# Autodesk Inventor assembly: LINEAR_INTAKE_ASSY
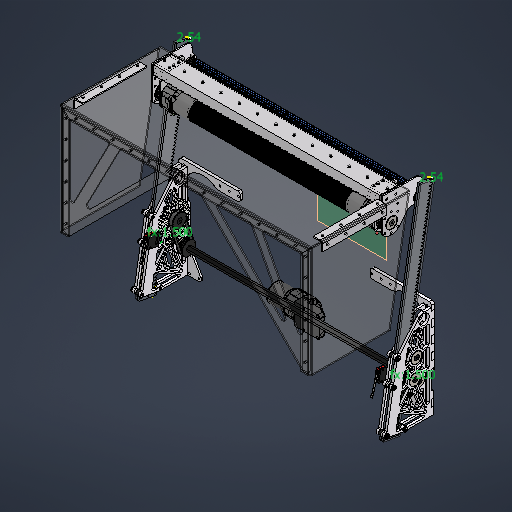
[picture p0: Inventor's stored thumbnail of the model, 512x512]
Saved by Autodesk Inventor 2026 (Build 300175000, 175)
## iProperties
Created: 2026-04-01
Part Number: LINEAR_INTAKE_ASSY
Document SubType Name: Assembly
Designer: 4aida
Mass: 10797 g
Surface Area: 25753.5 cm^2
Volume: 4543.31 cm^3
Density: 2.37645 g/cm^3
Author: 4aida
## Documents named in this file (44)
- C:\Users\littl\OneDrive\Documents\GitHub\2026-Robot-Mechanical\LINEAR_INTAKE\LINEAR_INTAKE_ASSY.iam
- C:\Users\littl\OneDrive\Documents\GitHub\2026-Robot-Mechanical\LINEAR_INTAKE\0.5_Jack_Shaft.ipt
- C:\Users\littl\OneDrive\Documents\GitHub\2026-Robot-Mechanical\#1_CAD Library\Electronics\CONTROLS,SPARK_FLEX.ipt
- C:\Users\littl\OneDrive\Documents\GitHub\2026-Robot-Mechanical\#1_CAD Library\Motors\MOTOR,REV,NEO,VORTEX.ipt
- C:\Users\littl\OneDrive\Documents\GitHub\2026-Robot-Mechanical\LINEAR_INTAKE\RACK_LINEARINTAKE.ipt
- C:\Users\littl\OneDrive\Documents\GitHub\2026-Robot-Mechanical\LINEAR_INTAKE\10DP_Pinion Gear.iam
- C:\Users\littl\OneDrive\Documents\GitHub\2026-Robot-Mechanical\#1_CAD Library\Power Transmission\Bearings\PURCHASED,HEX_BEARING.ipt
- C:\Users\littl\OneDrive\Documents\GitHub\2026-Robot-Mechanical\LINEAR_INTAKE\INTAKE_OUTSIDE_PLATE.ipt
- C:\Users\littl\OneDrive\Documents\GitHub\2026-Robot-Mechanical\LINEAR_INTAKE\RACK_GUIDES.ipt
- C:\Users\littl\OneDrive\Documents\GitHub\2026-Robot-Mechanical\LINEAR_INTAKE\CAST,2inOD,ROLLER.ipt
- C:\Users\littl\OneDrive\Documents\GitHub\2026-Robot-Mechanical\LINEAR_INTAKE\10dp_Ratio_Gears_INTAKE.iam
- C:\Users\littl\OneDrive\Documents\GitHub\2026-Robot-Mechanical\LINEAR_INTAKE\INTAKE_EXT_PULLYS.ipt
- C:\Users\littl\OneDrive\Documents\GitHub\2026-Robot-Mechanical\LINEAR_INTAKE\55t_Belt.ipt
- C:\Users\littl\OneDrive\Documents\GitHub\2026-Robot-Mechanical\LINEAR_INTAKE\12mm_OD_BEARING.ipt
- C:\Users\littl\OneDrive\Documents\GitHub\2026-Robot-Mechanical\LINEAR_INTAKE\fastenal_1140891.ipt
- C:\Users\littl\OneDrive\Documents\GitHub\2026-Robot-Mechanical\LINEAR_INTAKE\SINGLE_BEARING_SPACER.ipt
- C:\Users\littl\OneDrive\Documents\GitHub\2026-Robot-Mechanical\LINEAR_INTAKE\double_BEARING_SPACER.ipt
- C:\Users\littl\OneDrive\Documents\GitHub\2026-Robot-Mechanical\LINEAR_INTAKE\INTAKE_SWERVE_MOUNT.ipt
- C:\Users\littl\OneDrive\Documents\GitHub\2026-Robot-Mechanical\LINEAR_INTAKE\MOUTER_MOUNT_INTAKE.ipt
- C:\Users\littl\OneDrive\Documents\GitHub\2026-Robot-Mechanical\LINEAR_INTAKE\INTAKE_INSIDE_PLATE.ipt
- C:\Users\littl\OneDrive\Documents\GitHub\2026-Robot-Mechanical\LINEAR_INTAKE\INTAKE_BACK_MOUNT_PLATE.ipt
- C:\Users\littl\OneDrive\Documents\GitHub\2026-Robot-Mechanical\LINEAR_INTAKE\PULLY_HEX_SHAFT_INTAKE.ipt
- C:\Users\littl\OneDrive\Documents\GitHub\2026-Robot-Mechanical\LINEAR_INTAKE\PINION_SHAFT_INTAKE.ipt
- C:\Users\littl\OneDrive\Documents\GitHub\2026-Robot-Mechanical\LINEAR_INTAKE\TETHLON_TAPE.ipt
- C:\Users\littl\OneDrive\Documents\GitHub\2026-Robot-Mechanical\LINEAR_INTAKE\PINION_SPACER_INTAKE.ipt
- C:\Users\littl\OneDrive\Documents\GitHub\2026-Robot-Mechanical\LINEAR_INTAKE\PULLY_SPACER_INTAKE.ipt
- C:\Users\littl\OneDrive\Documents\GitHub\2026-Robot-Mechanical\LINEAR_INTAKE\1.25IN Roller.iam
- C:\Users\littl\OneDrive\Documents\GitHub\2026-Robot-Mechanical\LINEAR_INTAKE\CRASH_BAR_INTAKE.ipt
- C:\Users\littl\OneDrive\Documents\GitHub\2026-Robot-Mechanical\LINEAR_INTAKE\TUBE_PLUGS.ipt
- C:\Users\littl\OneDrive\Documents\GitHub\2026-Robot-Mechanical\#1_CAD Library\Electronics\CONTROLS,LIMIT_SWITCH,VEX.iam
- C:\Users\littl\OneDrive\Documents\GitHub\2026-Robot-Mechanical\LINEAR_INTAKE\INSIDE_INTAKE_PLATE.ipt
- C:\Users\littl\OneDrive\Documents\GitHub\2026-Robot-Mechanical\LINEAR_INTAKE\FRONT_INTAKE_LEXAN.ipt
- C:\Users\littl\OneDrive\Documents\GitHub\2026-Robot-Mechanical\LINEAR_INTAKE\SIDE_INTAKE_LEXAN.ipt
- C:\Users\littl\OneDrive\Documents\GitHub\2026-Robot-Mechanical\LINEAR_INTAKE\SIDE_INTAKE_LEXAN_MIR.ipt
- C:\Users\littl\OneDrive\Documents\GitHub\2026-Robot-Mechanical\LINEAR_INTAKE\TOP_INTAKE_LEXAN.ipt
- C:\Users\littl\OneDrive\Documents\GitHub\2026-Robot-Mechanical\LINEAR_INTAKE\LEXAN_CORNER_MOUNT.ipt
- C:\Users\littl\OneDrive\Documents\GitHub\2026-Robot-Mechanical\LINEAR_INTAKE\0.5_Bottom_INTAKE_SHAFT.ipt
- C:\Users\littl\OneDrive\Documents\GitHub\2026-Robot-Mechanical\LINEAR_INTAKE\INTAKE_DRIVER_PULLY.ipt
- C:\Users\littl\OneDrive\Documents\GitHub\2026-Robot-Mechanical\LINEAR_INTAKE\INTAKE_DRIVEN_PULLY.ipt
- C:\Users\littl\OneDrive\Documents\GitHub\2026-Robot-Mechanical\LINEAR_INTAKE\CUT_1.25_Roller.ipt
- C:\Users\littl\OneDrive\Documents\GitHub\2026-Robot-Mechanical\LINEAR_INTAKE\INSIDE_INTAKE_PLATE_MOTOR_MOUNT.ipt
- C:\Users\littl\OneDrive\Documents\GitHub\2026-Robot-Mechanical\LINEAR_INTAKE\CUT_2in_Roller.ipt
- C:\Users\littl\OneDrive\Documents\GitHub\2026-Robot-Mechanical\#1_CAD Library\Building Materials\Fasteners\Bolts\PURCHASED,10-32x0.5in,BUTTONHEAD,BOLT.ipt
- C:\Users\littl\OneDrive\Documents\GitHub\2026-Robot-Mechanical\LINEAR_INTAKE\INSIDE_INTAKE_PLATE_MOTOR_MOUNT_MIR.ipt
## Components (128 placed, 43 different names)
1. RACK_LINEARINTAKE:1 — Mate:149, Mate:230
2. 10DP_Pinion Gear:1 [sub-assembly] — Mate:19, Mate:201
3. INTAKE_OUTSIDE_PLATE:1 — Mate:66, Mate:67, Insert:3, Mate:121, Mate:122, Mate:123, Mate:124, Mate:125, Mate:126, Mate:128, Mate:129, Insert:4, Insert:5, Insert:6, Insert:7, Insert:8, Insert:9, Flush:27, Flush:28, Mate:169, Flush:31, Flush:39, Mate:200, Flush:40
4. INTAKE_OUTSIDE_PLATE:2 — Flush:18, Mate:60, Mate:63, Insert:1, Mate:131, Flush:30, Insert:21, Insert:22, Insert:23, Insert:24, Insert:25, Insert:27, Mate:171, Mate:174, Flush:37, Mate:196, Mate:198, Flush:42, Mate:316, Mate:317, Angle:9
5. RACK_LINEARINTAKE:2
6. 10DP_Pinion Gear:2 [sub-assembly] — Mate:19, Mate:195
7. RACK_GUIDES:1 — Mate:272, Angle:5, Flush:56, Mate:330
8. RACK_GUIDES:4 — Flush:18, Mate:196
9. PURCHASED,HEX_BEARING:3 — Mate:60, Mate:63, Mate:194, Mate:195, Mate:203, Mate:204
10. PURCHASED,HEX_BEARING:4 — Mate:106, Mate:177, Mate:178, Mate:192
11. PURCHASED,HEX_BEARING:5 — Mate:96, Mate:154, Mate:157
12. PURCHASED,HEX_BEARING:6 — Mate:66, Mate:67, Mate:189, Flush:34, Mate:190, Mate:202
13. PURCHASED,HEX_BEARING:7 — Mate:107, Mate:115, Mate:176, Mate:179, Mate:180, Mate:185
14. PURCHASED,HEX_BEARING:10 — Insert:1, Mate:184
15. PURCHASED,HEX_BEARING:11 — Mate:94, Mate:95, Mate:155, Mate:156
16. PURCHASED,HEX_BEARING:12 — Insert:3, Mate:188
17. 10dp_Ratio_Gears_INTAKE:3 [sub-assembly] — Mate:94, Mate:95, Mate:96, Mate:97, Mate:98, Mate:154, Mate:191
18. INTAKE_EXT_PULLYS:5 — Mate:97, Mate:98, Flush:33, Mate:186, Mate:187, Mate:319
19. 10dp_Ratio_Gears_INTAKE:4 [sub-assembly] — Mate:106, Mate:107, Mate:108, Mate:109, Flush:35, Mate:193
20. INTAKE_EXT_PULLYS:7 — Mate:108, Mate:109, Mate:115, Flush:32, Mate:183
21. 12mm_OD_BEARING:1 — Mate:121, Mate:124, Insert:13
22. 12mm_OD_BEARING:2 — Mate:119, Mate:120
23. 12mm_OD_BEARING:3 — Mate:125, Insert:11
24. 12mm_OD_BEARING:4 — Mate:122, Mate:123, Insert:15
25. 12mm_OD_BEARING:5 — Mate:119, Mate:120, Insert:10
26. 12mm_OD_BEARING:6 — Mate:126, Insert:12
27. 12mm_OD_BEARING:12 — Mate:128, Mate:129, Insert:14
28. fastenal_1140891:1 — Insert:4
29. fastenal_1140891:2 — Insert:5
30. fastenal_1140891:3 — Insert:8
31. fastenal_1140891:4 — Insert:9
32. fastenal_1140891:5 — Insert:7
33. fastenal_1140891:6 — Insert:6
34. SINGLE_BEARING_SPACER:3 — Insert:10
35. double_BEARING_SPACER:1 — Insert:11
36. double_BEARING_SPACER:2 — Insert:15
37. double_BEARING_SPACER:3 — Insert:12
38. double_BEARING_SPACER:4 — Insert:13
39. double_BEARING_SPACER:5 — Insert:14
40. INTAKE_SWERVE_MOUNT:1 — Flush:27, Flush:28, Flush:29, Mate:150, Mate:318
41. INTAKE_SWERVE_MOUNT:2 — Mate:131, Flush:29, Flush:30, Mate:172, Mate:181
42. 12mm_OD_BEARING:13 — Mate:135, Mate:136
43. fastenal_1140891:7 — Mate:135, Mate:136, Insert:24
44. double_BEARING_SPACER:6
45. 12mm_OD_BEARING:14
46. fastenal_1140891:8 — Insert:25
47. double_BEARING_SPACER:7
48. 12mm_OD_BEARING:15
49. fastenal_1140891:9 — Insert:23
50. double_BEARING_SPACER:8
51. 12mm_OD_BEARING:16
52. fastenal_1140891:10 — Insert:21
53. double_BEARING_SPACER:9
54. 12mm_OD_BEARING:17
55. fastenal_1140891:11 — Insert:22
56. double_BEARING_SPACER:10
57. 12mm_OD_BEARING:18
58. 12mm_OD_BEARING:19 — Mate:147
59. fastenal_1140891:12 — Mate:147, Mate:148, Insert:27
60. SINGLE_BEARING_SPACER:4 — Mate:148
61. INTAKE_INSIDE_PLATE:1 — Mate:149, Mate:150, Mate:155, Mate:156, Mate:157, Mate:168, Flush:38, Mate:199, Flush:41, Mate:289, Mate:290, Mate:291, Mate:292, Mate:300, Mate:318
62. INTAKE_BACK_MOUNT_PLATE:1 — Mate:168, Mate:169, Flush:31
63. INTAKE_BACK_MOUNT_PLATE:2 — Mate:171, Mate:315, Mate:316, Mate:317
64. INTAKE_INSIDE_PLATE:3 — Mate:172, Mate:174, Mate:176, Mate:177, Mate:178, Mate:179, Mate:180, Mate:181, Flush:36, Mate:197, Flush:43, Mate:286, Mate:287, Mate:288, Insert:28, Angle:6
65. PULLY_HEX_SHAFT_INTAKE:1 — Flush:32, Mate:183, Mate:184, Mate:185
66. PULLY_HEX_SHAFT_INTAKE:2 — Flush:33, Mate:186, Mate:187, Mate:188
67. PINION_SHAFT_INTAKE:1 — Mate:189, Flush:34, Mate:190, Mate:191
68. PINION_SHAFT_INTAKE:2 — Mate:192, Flush:35, Mate:193, Mate:194
69. TETHLON_TAPE:1 — Flush:36, Mate:197, Flush:43
70. TETHLON_TAPE:2 — Flush:38, Mate:198, Flush:42
71. TETHLON_TAPE:3 — Flush:37, Mate:200, Flush:40
72. TETHLON_TAPE:4 — Flush:39, Mate:199, Flush:41
73. PINION_SPACER_INTAKE:1 — Mate:203, Mate:204
74. PINION_SPACER_INTAKE:2 — Mate:201, Mate:202
75. CRASH_BAR_INTAKE:1 — Mate:220, Mate:224, Mate:225, Mate:226, Mate:227, Mate:228, Mate:229, Mate:230, Mate:274, Flush:55, Mate:330, Mate:373, Mate:374, Mate:386
76. TUBE_PLUGS:1 — Mate:227, Mate:228, Mate:229, Mate:235, Mate:236, Mate:263
77. TUBE_PLUGS:2 — Mate:224, Mate:225, Mate:226, Mate:231, Mate:232, Mate:233
78. INSIDE_INTAKE_PLATE:1 — Mate:231, Mate:232, Mate:233, Mate:242, Mate:327, Mate:328, Mate:335, Insert:29, Angle:7, Mate:385
79. 1.25IN Roller:6 [sub-assembly] — Mate:242, Mate:253, Mate:254, Flush:49, Mate:370
80. INSIDE_INTAKE_PLATE:2 — Mate:235, Mate:236, Mate:263, Mate:325, Mate:326, Mate:337, Mate:338, Angle:8, Mate:383
81. CAST,2inOD,ROLLER:9 — Mate:264, Mate:267, Mate:379
82. 1.25IN Roller:7 [sub-assembly] — Mate:253, Mate:254, Mate:255, Mate:256, Flush:49, Flush:50, Flush:51
83. 1.25IN Roller:8 [sub-assembly] — Mate:255, Mate:256, Flush:50, Mate:257, Mate:258, Flush:51
84. 1.25IN Roller:9 [sub-assembly] — Mate:257, Mate:258, Mate:371
85. CAST,2inOD,ROLLER:10 — Mate:264, Mate:265, Mate:267, Mate:268
86. CAST,2inOD,ROLLER:11 — Mate:265, Mate:268, Mate:367, Mate:368, Mate:369, Mate:380
87. FRONT_INTAKE_LEXAN:2 — Mate:274, Flush:55, Flush:56, Mate:275, Mate:276, Flush:57, Mate:277, Flush:58, Mate:278, Flush:60, Mate:280, Mate:282, Mate:285, Angle:9
88. SIDE_INTAKE_LEXAN:1 — Mate:275, Mate:276, Flush:57, Mate:281
89. SIDE_INTAKE_LEXAN_MIR:1 — Mate:277, Flush:58, Mate:278, Mate:279, Flush:59, Mate:283, Mate:284
90. TOP_INTAKE_LEXAN:1 — Mate:279, Flush:59, Flush:60
91. LEXAN_CORNER_MOUNT:1 — Mate:280, Mate:281, Mate:285
92. LEXAN_CORNER_MOUNT:2 — Mate:282, Mate:283, Mate:284
93. CONTROLS,LIMIT_SWITCH,VEX:2 [sub-assembly] — Mate:286, Mate:287, Mate:288
94. CONTROLS,LIMIT_SWITCH,VEX:3 [sub-assembly] — Mate:289, Mate:290, Mate:291
95. PURCHASED,HEX_BEARING:16 — Mate:292, Mate:294, Mate:299, Mate:300, Flush:61, Mate:321
96. 55t_Belt:3 — Mate:294, Mate:295, Mate:296, Mate:319
97. INTAKE_EXT_PULLYS:10 — Mate:295, Mate:296, Mate:297, Mate:298, Mate:301, Mate:324
98. PULLY_SPACER_INTAKE:3 — Mate:297, Mate:298, Mate:299
99. 0.5_Jack_Shaft:4 — Mate:301, Mate:320, Flush:61, Mate:321, Mate:322, Flush:62, Mate:323, Mate:324
100. PURCHASED,HEX_BEARING:17 — Insert:28, Mate:320, Flush:62, Mate:323
101. INTAKE_EXT_PULLYS:11 — Mate:305, Mate:307, Mate:308, Mate:322
102. PULLY_SPACER_INTAKE:4 — Mate:305
103. 55t_Belt:4 — Mate:307, Mate:308
104. CONTROLS,SPARK_FLEX:6
105. MOTOR,REV,NEO,VORTEX:6
106. MOUTER_MOUNT_INTAKE:2 — Mate:315, Angle:6
107. PURCHASED,HEX_BEARING:18 — Mate:325, Mate:326, Flush:63, Mate:331, Mate:363, Mate:364, Mate:365, Mate:382
108. PURCHASED,HEX_BEARING:19 — Mate:327, Mate:328, Mate:359, Mate:360, Mate:361, Mate:384
109. 0.5_Bottom_INTAKE_SHAFT:1 — Flush:63, Mate:331, Mate:359, Mate:362, Mate:364, Mate:366
110. CONTROLS,SPARK_FLEX:7 — Mate:356, Angle:7, Mate:388
111. MOTOR,REV,NEO,VORTEX:7 — Mate:357, Mate:379, Mate:387
112. 0.5_Bottom_INTAKE_SHAFT:2 — Mate:335, Flush:64, Mate:336, Mate:339, Mate:347, Mate:348, Mate:353, Mate:354, Mate:367, Mate:368, Mate:369
113. PURCHASED,HEX_BEARING:20 — Insert:29, Flush:64, Mate:336, Mate:343, Mate:344, Mate:350
114. PURCHASED,HEX_BEARING:21 — Mate:337, Mate:338, Mate:339, Mate:345, Mate:346
115. CONTROLS,SPARK_FLEX:8 — Mate:355, Angle:8, Mate:375
116. MOTOR,REV,NEO,VORTEX:8 — Mate:358, Mate:381
117. INTAKE_DRIVER_PULLY:1 — Mate:343, Mate:344, Mate:348, Mate:349
118. INTAKE_DRIVER_PULLY:2 — Mate:345, Mate:346, Mate:347, Mate:351, Mate:352
119. PURCHASED,HEX_BEARING:22 — Mate:349, Mate:350, Mate:354, Mate:356, Mate:357
120. PURCHASED,HEX_BEARING:23 — Mate:351, Mate:352, Mate:353, Mate:355, Mate:358
121. INTAKE_DRIVEN_PULLY:1 — Mate:360, Mate:361, Mate:362, Mate:370
122. INTAKE_DRIVEN_PULLY:2 — Mate:363, Mate:365, Mate:366, Mate:372
123. CUT_1.25_Roller:1 — Mate:371, Mate:372
124. INSIDE_INTAKE_PLATE_MOTOR_MOUNT:1 — Mate:373, Mate:374, Mate:375
125. CUT_2in_Roller:1 — Mate:380, Mate:381
126. PURCHASED,10-32x0.5in,BUTTONHEAD,BOLT:1 — Mate:382, Mate:383
127. PURCHASED,10-32x0.5in,BUTTONHEAD,BOLT:2 — Mate:384, Mate:385
128. INSIDE_INTAKE_PLATE_MOTOR_MOUNT_MIR:1 — Mate:386, Mate:387, Mate:388
## Relationships (290: Mate 217, Flush 40, Insert 28, Angle 5)
- [Flush]: RACK_LINEARINTAKE:1 ↔ 10DP_Pinion Gear:1
- [Flush] (6 mm): RACK_LINEARINTAKE:1 ↔ INTAKE_OUTSIDE_PLATE:1
- [Mate] (5.2705 mm): RACK_LINEARINTAKE:1 ↔ INTAKE_OUTSIDE_PLATE:1
- [Flush]: RACK_LINEARINTAKE:2 ↔ 10DP_Pinion Gear:2
- [Flush]: RACK_LINEARINTAKE:1 ↔ RACK_LINEARINTAKE:2
- [Flush]: RACK_LINEARINTAKE:1 ↔ RACK_LINEARINTAKE:2
- Mate:19: 10DP_Pinion Gear:1 ↔ 10DP_Pinion Gear:2
- [Mate]: RACK_LINEARINTAKE:1 ↔ RACK_GUIDES:1
- [Mate]: RACK_LINEARINTAKE:2 ↔ RACK_GUIDES:4
- [Flush]: RACK_LINEARINTAKE:2 ↔ RACK_GUIDES:4
- [Flush]: RACK_LINEARINTAKE:2 ↔ RACK_GUIDES:4
- [Flush]: RACK_LINEARINTAKE:1 ↔ RACK_GUIDES:1
- [Flush]: RACK_LINEARINTAKE:1 ↔ RACK_GUIDES:1
- Flush:18: INTAKE_OUTSIDE_PLATE:2 ↔ RACK_GUIDES:4
- Mate:60: INTAKE_OUTSIDE_PLATE:2 ↔ PURCHASED,HEX_BEARING:3
- Mate:63: INTAKE_OUTSIDE_PLATE:2 ↔ PURCHASED,HEX_BEARING:3
- Mate:66: INTAKE_OUTSIDE_PLATE:1 ↔ PURCHASED,HEX_BEARING:6
- Mate:67: INTAKE_OUTSIDE_PLATE:1 ↔ PURCHASED,HEX_BEARING:6
- Insert:1: INTAKE_OUTSIDE_PLATE:2 ↔ PURCHASED,HEX_BEARING:10
- Insert:3: INTAKE_OUTSIDE_PLATE:1 ↔ PURCHASED,HEX_BEARING:12
- Mate:94: PURCHASED,HEX_BEARING:11 ↔ 10dp_Ratio_Gears_INTAKE:3
- Mate:95: PURCHASED,HEX_BEARING:11 ↔ 10dp_Ratio_Gears_INTAKE:3
- Mate:96: PURCHASED,HEX_BEARING:5 ↔ 10dp_Ratio_Gears_INTAKE:3
- Mate:97: 10dp_Ratio_Gears_INTAKE:3 ↔ INTAKE_EXT_PULLYS:5
- Mate:98: 10dp_Ratio_Gears_INTAKE:3 ↔ INTAKE_EXT_PULLYS:5
- Mate:106: PURCHASED,HEX_BEARING:4 ↔ 10dp_Ratio_Gears_INTAKE:4
- Mate:107: PURCHASED,HEX_BEARING:7 ↔ 10dp_Ratio_Gears_INTAKE:4
- Mate:108: 10dp_Ratio_Gears_INTAKE:4 ↔ INTAKE_EXT_PULLYS:7
- Mate:109: 10dp_Ratio_Gears_INTAKE:4 ↔ INTAKE_EXT_PULLYS:7
- Mate:115: PURCHASED,HEX_BEARING:7 ↔ INTAKE_EXT_PULLYS:7
- Mate:119: 12mm_OD_BEARING:2 ↔ 12mm_OD_BEARING:5
- Mate:120: 12mm_OD_BEARING:2 ↔ 12mm_OD_BEARING:5
- Mate:121: INTAKE_OUTSIDE_PLATE:1 ↔ 12mm_OD_BEARING:1
- Mate:122: INTAKE_OUTSIDE_PLATE:1 ↔ 12mm_OD_BEARING:4
- Mate:123: INTAKE_OUTSIDE_PLATE:1 ↔ 12mm_OD_BEARING:4
- Mate:124: INTAKE_OUTSIDE_PLATE:1 ↔ 12mm_OD_BEARING:1
- Mate:125: INTAKE_OUTSIDE_PLATE:1 ↔ 12mm_OD_BEARING:3
- Mate:126: INTAKE_OUTSIDE_PLATE:1 ↔ 12mm_OD_BEARING:6
- Mate:128: INTAKE_OUTSIDE_PLATE:1 ↔ 12mm_OD_BEARING:12
- Mate:129: INTAKE_OUTSIDE_PLATE:1 ↔ 12mm_OD_BEARING:12
- Insert:4: INTAKE_OUTSIDE_PLATE:1 ↔ fastenal_1140891:1
- Insert:5: INTAKE_OUTSIDE_PLATE:1 ↔ fastenal_1140891:2
- Insert:6: INTAKE_OUTSIDE_PLATE:1 ↔ fastenal_1140891:6
- Insert:7: INTAKE_OUTSIDE_PLATE:1 ↔ fastenal_1140891:5
- Insert:8: INTAKE_OUTSIDE_PLATE:1 ↔ fastenal_1140891:3
- Insert:9: INTAKE_OUTSIDE_PLATE:1 ↔ fastenal_1140891:4
- Insert:10: 12mm_OD_BEARING:5 ↔ SINGLE_BEARING_SPACER:3
- Insert:11: 12mm_OD_BEARING:3 ↔ double_BEARING_SPACER:1
- Insert:12: 12mm_OD_BEARING:6 ↔ double_BEARING_SPACER:3
- Insert:13: 12mm_OD_BEARING:1 ↔ double_BEARING_SPACER:4
- Insert:14: 12mm_OD_BEARING:12 ↔ double_BEARING_SPACER:5
- Insert:15: 12mm_OD_BEARING:4 ↔ double_BEARING_SPACER:2
- Flush:27: INTAKE_OUTSIDE_PLATE:1 ↔ INTAKE_SWERVE_MOUNT:1
- Flush:28 (-12.2199 mm): INTAKE_OUTSIDE_PLATE:1 ↔ INTAKE_SWERVE_MOUNT:1
- Mate:131: INTAKE_OUTSIDE_PLATE:2 ↔ INTAKE_SWERVE_MOUNT:2
- Flush:29: INTAKE_SWERVE_MOUNT:1 ↔ INTAKE_SWERVE_MOUNT:2
- Flush:30: INTAKE_OUTSIDE_PLATE:2 ↔ INTAKE_SWERVE_MOUNT:2
- [Insert]: 12mm_OD_BEARING:13 ↔ double_BEARING_SPACER:6
- Mate:135 (6.35 mm): 12mm_OD_BEARING:13 ↔ fastenal_1140891:7
- Mate:136: 12mm_OD_BEARING:13 ↔ fastenal_1140891:7
- [Insert]: 12mm_OD_BEARING:14 ↔ double_BEARING_SPACER:7
- [Mate] (6.35 mm): 12mm_OD_BEARING:14 ↔ fastenal_1140891:8
- [Mate]: 12mm_OD_BEARING:14 ↔ fastenal_1140891:8
- [Insert]: 12mm_OD_BEARING:15 ↔ double_BEARING_SPACER:8
- [Mate] (6.35 mm): 12mm_OD_BEARING:15 ↔ fastenal_1140891:9
- [Mate]: 12mm_OD_BEARING:15 ↔ fastenal_1140891:9
- [Insert]: 12mm_OD_BEARING:16 ↔ double_BEARING_SPACER:9
- [Mate] (6.35 mm): 12mm_OD_BEARING:16 ↔ fastenal_1140891:10
- [Mate]: 12mm_OD_BEARING:16 ↔ fastenal_1140891:10
- [Insert]: 12mm_OD_BEARING:17 ↔ double_BEARING_SPACER:10
- [Mate] (6.35 mm): 12mm_OD_BEARING:17 ↔ fastenal_1140891:11
- [Mate]: 12mm_OD_BEARING:17 ↔ fastenal_1140891:11
- Insert:21: INTAKE_OUTSIDE_PLATE:2 ↔ fastenal_1140891:10
- Insert:22: INTAKE_OUTSIDE_PLATE:2 ↔ fastenal_1140891:11
- Insert:23: INTAKE_OUTSIDE_PLATE:2 ↔ fastenal_1140891:9
- Insert:24: INTAKE_OUTSIDE_PLATE:2 ↔ fastenal_1140891:7
- Insert:25: INTAKE_OUTSIDE_PLATE:2 ↔ fastenal_1140891:8
- [Mate]: 12mm_OD_BEARING:18 ↔ 12mm_OD_BEARING:19
- [Mate]: 12mm_OD_BEARING:18 ↔ 12mm_OD_BEARING:19
- [Insert]: 12mm_OD_BEARING:19 ↔ SINGLE_BEARING_SPACER:4
- Mate:147: 12mm_OD_BEARING:19 ↔ fastenal_1140891:12
- Mate:148 (6.35 mm): fastenal_1140891:12 ↔ SINGLE_BEARING_SPACER:4
- Insert:27: INTAKE_OUTSIDE_PLATE:2 ↔ fastenal_1140891:12
- Mate:149 (0.508 mm): RACK_LINEARINTAKE:1 ↔ INTAKE_INSIDE_PLATE:1
- Mate:150: INTAKE_SWERVE_MOUNT:1 ↔ INTAKE_INSIDE_PLATE:1
- Mate:154: PURCHASED,HEX_BEARING:5 ↔ 10dp_Ratio_Gears_INTAKE:3
- Mate:155: PURCHASED,HEX_BEARING:11 ↔ INTAKE_INSIDE_PLATE:1
- Mate:156: PURCHASED,HEX_BEARING:11 ↔ INTAKE_INSIDE_PLATE:1
- Mate:157: PURCHASED,HEX_BEARING:5 ↔ INTAKE_INSIDE_PLATE:1
- Mate:168: INTAKE_INSIDE_PLATE:1 ↔ INTAKE_BACK_MOUNT_PLATE:1
- Mate:169: INTAKE_OUTSIDE_PLATE:1 ↔ INTAKE_BACK_MOUNT_PLATE:1
- Flush:31: INTAKE_OUTSIDE_PLATE:1 ↔ INTAKE_BACK_MOUNT_PLATE:1
- Mate:171: INTAKE_OUTSIDE_PLATE:2 ↔ INTAKE_BACK_MOUNT_PLATE:2
- Mate:172: INTAKE_SWERVE_MOUNT:2 ↔ INTAKE_INSIDE_PLATE:3
- Mate:174: INTAKE_OUTSIDE_PLATE:2 ↔ INTAKE_INSIDE_PLATE:3
- Mate:176: PURCHASED,HEX_BEARING:7 ↔ INTAKE_INSIDE_PLATE:3
- Mate:177: PURCHASED,HEX_BEARING:4 ↔ INTAKE_INSIDE_PLATE:3
- Mate:178: PURCHASED,HEX_BEARING:4 ↔ INTAKE_INSIDE_PLATE:3
- Mate:179: PURCHASED,HEX_BEARING:7 ↔ INTAKE_INSIDE_PLATE:3
- Mate:180: PURCHASED,HEX_BEARING:7 ↔ INTAKE_INSIDE_PLATE:3
- Mate:181: INTAKE_SWERVE_MOUNT:2 ↔ INTAKE_INSIDE_PLATE:3
- Flush:32: INTAKE_EXT_PULLYS:7 ↔ PULLY_HEX_SHAFT_INTAKE:1
- Mate:183: INTAKE_EXT_PULLYS:7 ↔ PULLY_HEX_SHAFT_INTAKE:1
- Mate:184: PURCHASED,HEX_BEARING:10 ↔ PULLY_HEX_SHAFT_INTAKE:1
- Mate:185: PURCHASED,HEX_BEARING:7 ↔ PULLY_HEX_SHAFT_INTAKE:1
- Flush:33: INTAKE_EXT_PULLYS:5 ↔ PULLY_HEX_SHAFT_INTAKE:2
- Mate:186: INTAKE_EXT_PULLYS:5 ↔ PULLY_HEX_SHAFT_INTAKE:2
- Mate:187: INTAKE_EXT_PULLYS:5 ↔ PULLY_HEX_SHAFT_INTAKE:2
- Mate:188: PURCHASED,HEX_BEARING:12 ↔ PULLY_HEX_SHAFT_INTAKE:2
- Mate:189: PURCHASED,HEX_BEARING:6 ↔ PINION_SHAFT_INTAKE:1
- Flush:34: PURCHASED,HEX_BEARING:6 ↔ PINION_SHAFT_INTAKE:1
- Mate:190: PURCHASED,HEX_BEARING:6 ↔ PINION_SHAFT_INTAKE:1
- Mate:191: 10dp_Ratio_Gears_INTAKE:3 ↔ PINION_SHAFT_INTAKE:1
- Mate:192: PURCHASED,HEX_BEARING:4 ↔ PINION_SHAFT_INTAKE:2
- Flush:35: 10dp_Ratio_Gears_INTAKE:4 ↔ PINION_SHAFT_INTAKE:2
- Mate:193: 10dp_Ratio_Gears_INTAKE:4 ↔ PINION_SHAFT_INTAKE:2
- Mate:194: PURCHASED,HEX_BEARING:3 ↔ PINION_SHAFT_INTAKE:2
- Flush:36: INTAKE_INSIDE_PLATE:3 ↔ TETHLON_TAPE:1
- Flush:37: INTAKE_OUTSIDE_PLATE:2 ↔ TETHLON_TAPE:3
- Flush:38: INTAKE_INSIDE_PLATE:1 ↔ TETHLON_TAPE:2
- Flush:39: INTAKE_OUTSIDE_PLATE:1 ↔ TETHLON_TAPE:4
- Mate:195: 10DP_Pinion Gear:2 ↔ PURCHASED,HEX_BEARING:3
- Mate:196 (0.508 mm): INTAKE_OUTSIDE_PLATE:2 ↔ RACK_GUIDES:4
- Mate:197: INTAKE_INSIDE_PLATE:3 ↔ TETHLON_TAPE:1
- Mate:198: INTAKE_OUTSIDE_PLATE:2 ↔ TETHLON_TAPE:2
- Mate:199: INTAKE_INSIDE_PLATE:1 ↔ TETHLON_TAPE:4
- Mate:200: INTAKE_OUTSIDE_PLATE:1 ↔ TETHLON_TAPE:3
- Flush:40: INTAKE_OUTSIDE_PLATE:1 ↔ TETHLON_TAPE:3
- Flush:41: INTAKE_INSIDE_PLATE:1 ↔ TETHLON_TAPE:4
- Flush:42: INTAKE_OUTSIDE_PLATE:2 ↔ TETHLON_TAPE:2
- Flush:43: INTAKE_INSIDE_PLATE:3 ↔ TETHLON_TAPE:1
- Mate:201: 10DP_Pinion Gear:1 ↔ PINION_SPACER_INTAKE:2
- Mate:202: PURCHASED,HEX_BEARING:6 ↔ PINION_SPACER_INTAKE:2
- Mate:203: PURCHASED,HEX_BEARING:3 ↔ PINION_SPACER_INTAKE:1
- Mate:204: PURCHASED,HEX_BEARING:3 ↔ PINION_SPACER_INTAKE:1
- Mate:220: CRASH_BAR_INTAKE:1
- Mate:224: CRASH_BAR_INTAKE:1 ↔ TUBE_PLUGS:2
- Mate:225: CRASH_BAR_INTAKE:1 ↔ TUBE_PLUGS:2
- Mate:226: CRASH_BAR_INTAKE:1 ↔ TUBE_PLUGS:2
- Mate:227: CRASH_BAR_INTAKE:1 ↔ TUBE_PLUGS:1
- Mate:228: CRASH_BAR_INTAKE:1 ↔ TUBE_PLUGS:1
- Mate:229: CRASH_BAR_INTAKE:1 ↔ TUBE_PLUGS:1
- Mate:230: RACK_LINEARINTAKE:1 ↔ CRASH_BAR_INTAKE:1
- Mate:231: TUBE_PLUGS:2 ↔ INSIDE_INTAKE_PLATE:1
- Mate:232: TUBE_PLUGS:2 ↔ INSIDE_INTAKE_PLATE:1
- Mate:233: TUBE_PLUGS:2 ↔ INSIDE_INTAKE_PLATE:1
- Mate:235: TUBE_PLUGS:1 ↔ INSIDE_INTAKE_PLATE:2
- Mate:236: TUBE_PLUGS:1 ↔ INSIDE_INTAKE_PLATE:2
- Mate:242: INSIDE_INTAKE_PLATE:1 ↔ 1.25IN Roller:6
- Mate:253: 1.25IN Roller:6 ↔ 1.25IN Roller:7
- Mate:254: 1.25IN Roller:6 ↔ 1.25IN Roller:7
- Mate:255: 1.25IN Roller:7 ↔ 1.25IN Roller:8
- Mate:256: 1.25IN Roller:7 ↔ 1.25IN Roller:8
- Flush:49: 1.25IN Roller:6 ↔ 1.25IN Roller:7
- Flush:50: 1.25IN Roller:7 ↔ 1.25IN Roller:8
- Mate:257: 1.25IN Roller:8 ↔ 1.25IN Roller:9
- Mate:258: 1.25IN Roller:8 ↔ 1.25IN Roller:9
- Flush:51: 1.25IN Roller:7 ↔ 1.25IN Roller:8
- Mate:263: TUBE_PLUGS:1 ↔ INSIDE_INTAKE_PLATE:2
- Mate:264: CAST,2inOD,ROLLER:9 ↔ CAST,2inOD,ROLLER:10
- Mate:265: CAST,2inOD,ROLLER:10 ↔ CAST,2inOD,ROLLER:11
- Mate:267: CAST,2inOD,ROLLER:9 ↔ CAST,2inOD,ROLLER:10
- Mate:268: CAST,2inOD,ROLLER:10 ↔ CAST,2inOD,ROLLER:11
- Mate:272: RACK_GUIDES:1
- Angle:5 (10 deg): RACK_GUIDES:1
- Mate:274: CRASH_BAR_INTAKE:1 ↔ FRONT_INTAKE_LEXAN:2
- Flush:55: CRASH_BAR_INTAKE:1 ↔ FRONT_INTAKE_LEXAN:2
- Flush:56 (-3.175 mm): RACK_GUIDES:1 ↔ FRONT_INTAKE_LEXAN:2
- Mate:275: FRONT_INTAKE_LEXAN:2 ↔ SIDE_INTAKE_LEXAN:1
- Mate:276: FRONT_INTAKE_LEXAN:2 ↔ SIDE_INTAKE_LEXAN:1
- Flush:57: FRONT_INTAKE_LEXAN:2 ↔ SIDE_INTAKE_LEXAN:1
- Mate:277: FRONT_INTAKE_LEXAN:2 ↔ SIDE_INTAKE_LEXAN_MIR:1
- Flush:58: FRONT_INTAKE_LEXAN:2 ↔ SIDE_INTAKE_LEXAN_MIR:1
- Mate:278: FRONT_INTAKE_LEXAN:2 ↔ SIDE_INTAKE_LEXAN_MIR:1
- Mate:279: SIDE_INTAKE_LEXAN_MIR:1 ↔ TOP_INTAKE_LEXAN:1
- Flush:59: SIDE_INTAKE_LEXAN_MIR:1 ↔ TOP_INTAKE_LEXAN:1
- Flush:60: FRONT_INTAKE_LEXAN:2 ↔ TOP_INTAKE_LEXAN:1
- Mate:280: FRONT_INTAKE_LEXAN:2 ↔ LEXAN_CORNER_MOUNT:1
- Mate:281: SIDE_INTAKE_LEXAN:1 ↔ LEXAN_CORNER_MOUNT:1
- Mate:282: FRONT_INTAKE_LEXAN:2 ↔ LEXAN_CORNER_MOUNT:2
- Mate:283: SIDE_INTAKE_LEXAN_MIR:1 ↔ LEXAN_CORNER_MOUNT:2
- Mate:284: SIDE_INTAKE_LEXAN_MIR:1 ↔ LEXAN_CORNER_MOUNT:2
- Mate:285: FRONT_INTAKE_LEXAN:2 ↔ LEXAN_CORNER_MOUNT:1
- Mate:286: INTAKE_INSIDE_PLATE:3 ↔ CONTROLS,LIMIT_SWITCH,VEX:2
- Mate:287 (-12.7 mm): INTAKE_INSIDE_PLATE:3 ↔ CONTROLS,LIMIT_SWITCH,VEX:2
- Mate:288: INTAKE_INSIDE_PLATE:3 ↔ CONTROLS,LIMIT_SWITCH,VEX:2
- Mate:289: INTAKE_INSIDE_PLATE:1 ↔ CONTROLS,LIMIT_SWITCH,VEX:3
- Mate:290: INTAKE_INSIDE_PLATE:1 ↔ CONTROLS,LIMIT_SWITCH,VEX:3
- Mate:291: INTAKE_INSIDE_PLATE:1 ↔ CONTROLS,LIMIT_SWITCH,VEX:3
- Mate:292: INTAKE_INSIDE_PLATE:1 ↔ PURCHASED,HEX_BEARING:16
- Mate:294: PURCHASED,HEX_BEARING:16 ↔ 55t_Belt:3
- Mate:295: 55t_Belt:3 ↔ INTAKE_EXT_PULLYS:10
- Mate:296: 55t_Belt:3 ↔ INTAKE_EXT_PULLYS:10
- Mate:297: INTAKE_EXT_PULLYS:10 ↔ PULLY_SPACER_INTAKE:3
- Mate:298: INTAKE_EXT_PULLYS:10 ↔ PULLY_SPACER_INTAKE:3
- Mate:299: PURCHASED,HEX_BEARING:16 ↔ PULLY_SPACER_INTAKE:3
- Mate:300: INTAKE_INSIDE_PLATE:1 ↔ PURCHASED,HEX_BEARING:16
- Mate:301: INTAKE_EXT_PULLYS:10 ↔ 0.5_Jack_Shaft:4
- [Mate]: PURCHASED,HEX_BEARING:17 ↔ INTAKE_EXT_PULLYS:11
- [Mate]: PURCHASED,HEX_BEARING:17 ↔ PULLY_SPACER_INTAKE:4
- [Mate]: PURCHASED,HEX_BEARING:17 ↔ PULLY_SPACER_INTAKE:4
- Insert:28: INTAKE_INSIDE_PLATE:3 ↔ PURCHASED,HEX_BEARING:17
- Mate:305: INTAKE_EXT_PULLYS:11 ↔ PULLY_SPACER_INTAKE:4
- Mate:307: INTAKE_EXT_PULLYS:11 ↔ 55t_Belt:4
- Mate:308: INTAKE_EXT_PULLYS:11 ↔ 55t_Belt:4
- [Mate]: CONTROLS,SPARK_FLEX:6 ↔ MOTOR,REV,NEO,VORTEX:6
- [Mate]: CONTROLS,SPARK_FLEX:6 ↔ MOTOR,REV,NEO,VORTEX:6
- [Mate]: CONTROLS,SPARK_FLEX:6 ↔ MOTOR,REV,NEO,VORTEX:6
- [Mate]: CONTROLS,SPARK_FLEX:6 ↔ MOUTER_MOUNT_INTAKE:2
- [Mate]: MOTOR,REV,NEO,VORTEX:6 ↔ MOUTER_MOUNT_INTAKE:2
- [Mate]: CONTROLS,SPARK_FLEX:6 ↔ MOUTER_MOUNT_INTAKE:2
- Mate:315 (3.175 mm): INTAKE_BACK_MOUNT_PLATE:2 ↔ MOUTER_MOUNT_INTAKE:2
- Mate:316: INTAKE_OUTSIDE_PLATE:2 ↔ INTAKE_BACK_MOUNT_PLATE:2
- Mate:317: INTAKE_OUTSIDE_PLATE:2 ↔ INTAKE_BACK_MOUNT_PLATE:2
- Angle:6 (0 deg): INTAKE_INSIDE_PLATE:3 ↔ MOUTER_MOUNT_INTAKE:2
- Mate:318: INTAKE_SWERVE_MOUNT:1 ↔ INTAKE_INSIDE_PLATE:1
- Mate:319: INTAKE_EXT_PULLYS:5 ↔ 55t_Belt:3
- Mate:320: 0.5_Jack_Shaft:4 ↔ PURCHASED,HEX_BEARING:17
- Flush:61: PURCHASED,HEX_BEARING:16 ↔ 0.5_Jack_Shaft:4
- Mate:321: PURCHASED,HEX_BEARING:16 ↔ 0.5_Jack_Shaft:4
- Mate:322: 0.5_Jack_Shaft:4 ↔ INTAKE_EXT_PULLYS:11
- Flush:62: 0.5_Jack_Shaft:4 ↔ PURCHASED,HEX_BEARING:17
- Mate:323: 0.5_Jack_Shaft:4 ↔ PURCHASED,HEX_BEARING:17
- Mate:324: INTAKE_EXT_PULLYS:10 ↔ 0.5_Jack_Shaft:4
- Mate:325: INSIDE_INTAKE_PLATE:2 ↔ PURCHASED,HEX_BEARING:18
- Mate:326: INSIDE_INTAKE_PLATE:2 ↔ PURCHASED,HEX_BEARING:18
- Mate:327: INSIDE_INTAKE_PLATE:1 ↔ PURCHASED,HEX_BEARING:19
- Mate:328: INSIDE_INTAKE_PLATE:1 ↔ PURCHASED,HEX_BEARING:19
- Mate:330 (-120.8143 mm): RACK_GUIDES:1 ↔ CRASH_BAR_INTAKE:1
- Flush:63: PURCHASED,HEX_BEARING:18 ↔ 0.5_Bottom_INTAKE_SHAFT:1
- Mate:331: PURCHASED,HEX_BEARING:18 ↔ 0.5_Bottom_INTAKE_SHAFT:1
- [Mate]: CONTROLS,SPARK_FLEX:7 ↔ MOTOR,REV,NEO,VORTEX:7
- [Mate]: CONTROLS,SPARK_FLEX:7 ↔ MOTOR,REV,NEO,VORTEX:7
- [Mate]: CONTROLS,SPARK_FLEX:7 ↔ MOTOR,REV,NEO,VORTEX:7
- Mate:335: INSIDE_INTAKE_PLATE:1 ↔ 0.5_Bottom_INTAKE_SHAFT:2
- Insert:29: INSIDE_INTAKE_PLATE:1 ↔ PURCHASED,HEX_BEARING:20
- Flush:64: 0.5_Bottom_INTAKE_SHAFT:2 ↔ PURCHASED,HEX_BEARING:20
- Mate:336: 0.5_Bottom_INTAKE_SHAFT:2 ↔ PURCHASED,HEX_BEARING:20
- Mate:337: INSIDE_INTAKE_PLATE:2 ↔ PURCHASED,HEX_BEARING:21
- Mate:338: INSIDE_INTAKE_PLATE:2 ↔ PURCHASED,HEX_BEARING:21
- Mate:339: 0.5_Bottom_INTAKE_SHAFT:2 ↔ PURCHASED,HEX_BEARING:21
- [Mate]: CONTROLS,SPARK_FLEX:8 ↔ MOTOR,REV,NEO,VORTEX:8
- [Mate]: CONTROLS,SPARK_FLEX:8 ↔ MOTOR,REV,NEO,VORTEX:8
- [Mate]: CONTROLS,SPARK_FLEX:8 ↔ MOTOR,REV,NEO,VORTEX:8
- Mate:343: PURCHASED,HEX_BEARING:20 ↔ INTAKE_DRIVER_PULLY:1
- Mate:344: PURCHASED,HEX_BEARING:20 ↔ INTAKE_DRIVER_PULLY:1
- Mate:345: PURCHASED,HEX_BEARING:21 ↔ INTAKE_DRIVER_PULLY:2
- Mate:346: PURCHASED,HEX_BEARING:21 ↔ INTAKE_DRIVER_PULLY:2
- Mate:347: 0.5_Bottom_INTAKE_SHAFT:2 ↔ INTAKE_DRIVER_PULLY:2
- Mate:348: 0.5_Bottom_INTAKE_SHAFT:2 ↔ INTAKE_DRIVER_PULLY:1
- Mate:349: INTAKE_DRIVER_PULLY:1 ↔ PURCHASED,HEX_BEARING:22
- Mate:350: PURCHASED,HEX_BEARING:20 ↔ PURCHASED,HEX_BEARING:22
- Mate:351: INTAKE_DRIVER_PULLY:2 ↔ PURCHASED,HEX_BEARING:23
- Mate:352: INTAKE_DRIVER_PULLY:2 ↔ PURCHASED,HEX_BEARING:23
- Mate:353: 0.5_Bottom_INTAKE_SHAFT:2 ↔ PURCHASED,HEX_BEARING:23
- Mate:354: 0.5_Bottom_INTAKE_SHAFT:2 ↔ PURCHASED,HEX_BEARING:22
- Mate:355: CONTROLS,SPARK_FLEX:8 ↔ PURCHASED,HEX_BEARING:23
- Mate:356: CONTROLS,SPARK_FLEX:7 ↔ PURCHASED,HEX_BEARING:22
- Mate:357: MOTOR,REV,NEO,VORTEX:7 ↔ PURCHASED,HEX_BEARING:22
- Mate:358: MOTOR,REV,NEO,VORTEX:8 ↔ PURCHASED,HEX_BEARING:23
- Mate:359: PURCHASED,HEX_BEARING:19 ↔ 0.5_Bottom_INTAKE_SHAFT:1
- Mate:360: PURCHASED,HEX_BEARING:19 ↔ INTAKE_DRIVEN_PULLY:1
- Mate:361: PURCHASED,HEX_BEARING:19 ↔ INTAKE_DRIVEN_PULLY:1
- Mate:362: 0.5_Bottom_INTAKE_SHAFT:1 ↔ INTAKE_DRIVEN_PULLY:1
- Mate:363: PURCHASED,HEX_BEARING:18 ↔ INTAKE_DRIVEN_PULLY:2
- Mate:364: PURCHASED,HEX_BEARING:18 ↔ 0.5_Bottom_INTAKE_SHAFT:1
- Mate:365: PURCHASED,HEX_BEARING:18 ↔ INTAKE_DRIVEN_PULLY:2
- Mate:366: 0.5_Bottom_INTAKE_SHAFT:1 ↔ INTAKE_DRIVEN_PULLY:2
- Mate:367: CAST,2inOD,ROLLER:11 ↔ 0.5_Bottom_INTAKE_SHAFT:2
- Mate:368: CAST,2inOD,ROLLER:11 ↔ 0.5_Bottom_INTAKE_SHAFT:2
- Mate:369: CAST,2inOD,ROLLER:11 ↔ 0.5_Bottom_INTAKE_SHAFT:2
- Angle:7 (90 deg): INSIDE_INTAKE_PLATE:1 ↔ CONTROLS,SPARK_FLEX:7
- Angle:8 (90 deg): INSIDE_INTAKE_PLATE:2 ↔ CONTROLS,SPARK_FLEX:8
- Mate:370: 1.25IN Roller:6 ↔ INTAKE_DRIVEN_PULLY:1
- Mate:371: 1.25IN Roller:9 ↔ CUT_1.25_Roller:1
- Mate:372: INTAKE_DRIVEN_PULLY:2 ↔ CUT_1.25_Roller:1
- Mate:373: CRASH_BAR_INTAKE:1 ↔ INSIDE_INTAKE_PLATE_MOTOR_MOUNT:1
- Mate:374: CRASH_BAR_INTAKE:1 ↔ INSIDE_INTAKE_PLATE_MOTOR_MOUNT:1
- Mate:375: CONTROLS,SPARK_FLEX:8 ↔ INSIDE_INTAKE_PLATE_MOTOR_MOUNT:1
- Mate:379: CAST,2inOD,ROLLER:9 ↔ MOTOR,REV,NEO,VORTEX:7
- Mate:380: CAST,2inOD,ROLLER:11 ↔ CUT_2in_Roller:1
- Mate:381: MOTOR,REV,NEO,VORTEX:8 ↔ CUT_2in_Roller:1
- Mate:382: PURCHASED,HEX_BEARING:18 ↔ PURCHASED,10-32x0.5in,BUTTONHEAD,BOLT:1
- Mate:383: INSIDE_INTAKE_PLATE:2 ↔ PURCHASED,10-32x0.5in,BUTTONHEAD,BOLT:1
- Mate:384: PURCHASED,HEX_BEARING:19 ↔ PURCHASED,10-32x0.5in,BUTTONHEAD,BOLT:2
- Mate:385: INSIDE_INTAKE_PLATE:1 ↔ PURCHASED,10-32x0.5in,BUTTONHEAD,BOLT:2
- Mate:386: CRASH_BAR_INTAKE:1 ↔ INSIDE_INTAKE_PLATE_MOTOR_MOUNT_MIR:1
- Mate:387: MOTOR,REV,NEO,VORTEX:7 ↔ INSIDE_INTAKE_PLATE_MOTOR_MOUNT_MIR:1
- Mate:388: CONTROLS,SPARK_FLEX:7 ↔ INSIDE_INTAKE_PLATE_MOTOR_MOUNT_MIR:1
- Angle:9 (0 deg): INTAKE_OUTSIDE_PLATE:2 ↔ FRONT_INTAKE_LEXAN:2
## Named parameters: d193_d174 = 0 mm, d265_d252 = 0 mm, d268_d265_d252 = 0 mm, d269_d266 = 6.35 mm, d270_d267 = 0 mm, d271_d265_d252 = 0 mm, d272_d266 = 6.35 mm, d273_d267 = 0 mm, d274_d265_d252 = 0 mm, d275_d266 = 6.35 mm, d276_d267 = 0 mm, d277_d265_d252 = 0 mm, d278_d266 = 6.35 mm, d279_d267 = 0 mm, d285_d250 = 0 mm, d286_d229 = 0 mm, d287_d230 = 0 mm, d493_d201 = 0 mm, d494_d361 = 0 mm, d495_d362 = 0 mm, d501_d262 = 0 mm, d502_d263 = 0 mm, d503_d264 = 0 mm, d504_d163_d8 = 0 mm, d505_d164_d9 = 0 mm, d506_d165_d10 = 0 mm, d534_d406_d72_d163_d8 = 0 mm, d535_d407_d73_d164_d9 = 0 mm, d536_d408_d74_d165_d10 = 0 mm, d544_d534_d406_d72_d163_d8 = 0 mm, d545_d535_d407_d73_d164_d9 = 0 mm, d546_d536_d408_d74_d165_d10 = 0 mm
